# Autodesk Inventor assembly: 横回転ユニット改
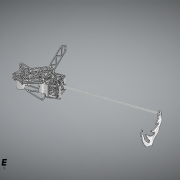
[picture p0: Inventor's stored thumbnail of the model, 180x180]
Saved by Autodesk Inventor 2020 (Build 240168000, 168)
## iProperties
Created: 2020-02-25
Part Number: 横回転ユニット改
Document SubType Name: Assembly
Designer: tanjihayato
Mass: 802.407 g
Surface Area: 1513.59 cm^2
Volume: 280.792 cm^3
Density: 2.85766 g/cm^3
Author: tanjihayato
## Documents named in this file (29)
- \\Mac\Home\Documents\Inventor\2019お遊び機体\横回転ユニット改.iam
- \\Mac\Home\Documents\Inventor\2019お遊び機体\横回転フレーム改.ipt
- \\Mac\Home\Documents\Inventor\2019お遊び機体\横回転フレーム改２.ipt
- \\Mac\Home\Documents\Inventor\2019お遊び機体\横回転フレーム改３.ipt
- \\Mac\Home\Documents\Inventor\2019お遊び機体\スペーサ　m3-l20.ipt
- \\Mac\Home\Documents\Inventor\2019お遊び機体\スペーサ　m3-l30.ipt
- \\Mac\Home\Documents\Inventor\2019お遊び機体\スペーサ　m3-l7.ipt
- \\Mac\Home\Documents\Inventor\2019お遊び機体\モーター(形だけ).ipt
- \\Mac\Home\Documents\Inventor\2019お遊び機体\横回転最終段.ipt
- \\Mac\Home\Documents\Inventor\2019お遊び機体\横回転最終段カム.ipt
- \\Mac\Home\Documents\Inventor\2019お遊び機体\横回転棒取り付けパーツ.ipt
- \\Mac\Home\Documents\Inventor\2019お遊び機体\横回転スライダー.ipt
- \\Mac\Home\Documents\Inventor\2019お遊び機体\ねじ皿　m3-l8.ipt
- \\Mac\Home\Documents\Inventor\2019お遊び機体\横回転フランジ付き軸.ipt
- \\Mac\Home\Documents\Inventor\2019お遊び機体\横回転シャフト.ipt
- \\Mac\Home\Documents\Inventor\2019お遊び機体\横回転フレーム改横.ipt
- \\Mac\Home\Documents\Inventor\2019お遊び機体\スペーサ　m3-l55.ipt
- \\Mac\Home\Documents\Inventor\2019お遊び機体\横回転首振りフレーム.ipt
- \\Mac\Home\Documents\Inventor\2019お遊び機体\横回転首振りフレーム２.ipt
- \\Mac\Home\Documents\Inventor\2019お遊び機体\スペーサ　m3-l12.ipt
- \\Mac\Home\Documents\Inventor\2019お遊び機体\アーム下板.ipt
- \\Mac\Home\Documents\Inventor\2019お遊び機体\スペーサ　m4-l45.ipt
- \\Mac\Home\Documents\Inventor\2019お遊び機体\横回転首振り駆動.ipt
- \\Mac\Home\Documents\Inventor\2019お遊び機体\フランジブッシュ　d8-D10-l5-f16.ipt
- \\Mac\Home\Documents\Inventor\2019お遊び機体\横回転鎌.ipt
- \\Mac\Home\Documents\Inventor\2019お遊び機体\m2z25.ipt
- \\Mac\Home\Documents\Inventor\2019お遊び機体\横回転首振り最終段カム.ipt
- \\Mac\Home\Documents\Inventor\2019お遊び機体\横回転カウンター根本.ipt
- \\Mac\Home\Documents\Inventor\2019お遊び機体\横回転首振りフレーム３.ipt
## Components (49 placed, 28 different names)
1. 横回転フレーム改:1 — 挿入:1, 挿入:2, 挿入:3, 挿入:4, 挿入:9, 挿入:10, 挿入:11, 挿入:12
2. 横回転フレーム改２:1 — 挿入:5, メイト:1, 挿入:7, 挿入:8, 挿入:14, メイト:3, メイト:4, メイト:5, メイト:6, メイト:7
3. 横回転フレーム改３:1 — 挿入:13, メイト:2
4. スペーサ　m3-l20:2 — 挿入:2, メイト:1
5. スペーサ　m3-l20:4 — 挿入:1, 挿入:5
6. スペーサ　m3-l30:1 — 挿入:4, メイト:2
7. スペーサ　m3-l30:2 — 挿入:3, 挿入:13
8. スペーサ　m3-l7:1 — 挿入:7
9. スペーサ　m3-l7:2 — 挿入:8
10. モーター(形だけ):1 — 挿入:9
11. モーター(形だけ):2 — 挿入:10
12. モーター(形だけ):3 — 挿入:11
13. モーター(形だけ):4 — 挿入:12
14. 横回転最終段:1 — 挿入:15, 挿入:23
15. 横回転最終段カム:1 — 挿入:14, メイト:3, 挿入:15, 挿入:16, 挿入:17, 挿入:25
16. 横回転棒取り付けパーツ:1 — 挿入:21, 挿入:22, 挿入:26
17. 横回転スライダー:1 — 挿入:21, 挿入:22, 挿入:24
18. ねじ皿　m3-l8:1 — 挿入:16
19. ねじ皿　m3-l8:2 — 挿入:17
20. 横回転フランジ付き軸:1 — 挿入:23, 挿入:24
21. 横回転フランジ付き軸:2 — 挿入:25
22. 横回転シャフト:1 — 挿入:26, 挿入:44
23. 横回転フレーム改横:1 — メイト:4, メイト:5
24. 横回転フレーム改横:2 — メイト:6, メイト:7, 挿入:27, 挿入:28, 挿入:29, 挿入:30, 挿入:42
25. スペーサ　m3-l55:1 — 挿入:30
26. スペーサ　m3-l55:2 — 挿入:29
27. スペーサ　m3-l55:3 — 挿入:27
28. スペーサ　m3-l55:4 — 挿入:28
29. 横回転首振りフレーム:1 — 挿入:35, メイト:11, 挿入:37, 挿入:38, 挿入:39, 挿入:40, 挿入:41, メイト:16, メイト:17, 挿入:47
30. 横回転首振りフレーム２:1 — メイト:8, メイト:9, メイト:10, 挿入:31, 挿入:32, 挿入:33, 挿入:34, 挿入:36, メイト:18, 挿入:48
31. スペーサ　m3-l12:1 — 挿入:33
32. スペーサ　m3-l12:2 — 挿入:31
33. スペーサ　m3-l12:3 — 挿入:34, 挿入:35
34. スペーサ　m3-l12:4 — 挿入:32, メイト:11
35. アーム下板:1 — メイト:8, メイト:9, メイト:10
36. スペーサ　m4-l45:1 — 挿入:36, メイト:12
37. スペーサ　m4-l45:2 — 挿入:38
38. スペーサ　m4-l45:3 — 挿入:37
39. モーター(形だけ):5 — 挿入:39
40. モーター(形だけ):6 — 挿入:40
41. 横回転首振り駆動:1 — 挿入:41, メイト:13, 挿入:43, 挿入:45, メイト:14
42. フランジブッシュ　d8-D10-l5-f16:1 — メイト:12, メイト:13
43. フランジブッシュ　d8-D10-l5-f16:2 — 挿入:42, 挿入:43
44. 横回転鎌:1 — 挿入:44
45. m2z25:1 — 挿入:46, メイト:15
46. 横回転首振り最終段カム:1 — 挿入:45, メイト:14, 挿入:46, メイト:15
47. 横回転カウンター根本:1 — メイト:16, メイト:17
48. 横回転首振りフレーム３:1 — 挿入:47, メイト:18
49. スペーサ　m3-l12:5 — 挿入:48
## Relationships (62: Insert 44, Mate 18)
- 挿入:1 [Insert]: 横回転フレーム改:1 ↔ スペーサ　m3-l20:4
- 挿入:2 [Insert]: 横回転フレーム改:1 ↔ スペーサ　m3-l20:2
- 挿入:3 [Insert]: 横回転フレーム改:1 ↔ スペーサ　m3-l30:2
- 挿入:4 [Insert]: 横回転フレーム改:1 ↔ スペーサ　m3-l30:1
- 挿入:5 [Insert]: 横回転フレーム改２:1 ↔ スペーサ　m3-l20:4
- メイト:1 [Mate]: 横回転フレーム改２:1 ↔ スペーサ　m3-l20:2
- 挿入:7 [Insert]: 横回転フレーム改２:1 ↔ スペーサ　m3-l7:1
- 挿入:8 [Insert]: 横回転フレーム改２:1 ↔ スペーサ　m3-l7:2
- 挿入:9 [Insert]: 横回転フレーム改:1 ↔ モーター(形だけ):1
- 挿入:10 [Insert]: 横回転フレーム改:1 ↔ モーター(形だけ):2
- 挿入:11 [Insert]: 横回転フレーム改:1 ↔ モーター(形だけ):3
- 挿入:12 [Insert]: 横回転フレーム改:1 ↔ モーター(形だけ):4
- 挿入:13 [Insert]: 横回転フレーム改３:1 ↔ スペーサ　m3-l30:2
- メイト:2 [Mate]: 横回転フレーム改３:1 ↔ スペーサ　m3-l30:1
- 挿入:14 [Insert]: 横回転フレーム改２:1 ↔ 横回転最終段カム:1
- メイト:3 [Mate]: 横回転フレーム改２:1 ↔ 横回転最終段カム:1
- 挿入:15 [Insert] (0.5 mm): 横回転最終段:1 ↔ 横回転最終段カム:1
- 挿入:16 [Insert]: 横回転最終段カム:1 ↔ ねじ皿　m3-l8:1
- 挿入:17 [Insert]: 横回転最終段カム:1 ↔ ねじ皿　m3-l8:2
- 挿入:21 [Insert]: 横回転棒取り付けパーツ:1 ↔ 横回転スライダー:1
- 挿入:22 [Insert]: 横回転棒取り付けパーツ:1 ↔ 横回転スライダー:1
- 挿入:23 [Insert]: 横回転最終段:1 ↔ 横回転フランジ付き軸:1
- 挿入:24 [Insert]: 横回転スライダー:1 ↔ 横回転フランジ付き軸:1
- 挿入:25 [Insert]: 横回転最終段カム:1 ↔ 横回転フランジ付き軸:2
- 挿入:26 [Insert]: 横回転棒取り付けパーツ:1 ↔ 横回転シャフト:1
- メイト:4 [Mate]: 横回転フレーム改２:1 ↔ 横回転フレーム改横:1
- メイト:5 [Mate]: 横回転フレーム改２:1 ↔ 横回転フレーム改横:1
- メイト:6 [Mate]: 横回転フレーム改２:1 ↔ 横回転フレーム改横:2
- メイト:7 [Mate]: 横回転フレーム改２:1 ↔ 横回転フレーム改横:2
- 挿入:27 [Insert]: 横回転フレーム改横:2 ↔ スペーサ　m3-l55:3
- 挿入:28 [Insert]: 横回転フレーム改横:2 ↔ スペーサ　m3-l55:4
- 挿入:29 [Insert]: 横回転フレーム改横:2 ↔ スペーサ　m3-l55:2
- 挿入:30 [Insert]: 横回転フレーム改横:2 ↔ スペーサ　m3-l55:1
- メイト:8 [Mate]: 横回転首振りフレーム２:1 ↔ アーム下板:1
- メイト:9 [Mate]: 横回転首振りフレーム２:1 ↔ アーム下板:1
- メイト:10 [Mate]: 横回転首振りフレーム２:1 ↔ アーム下板:1
- 挿入:31 [Insert]: 横回転首振りフレーム２:1 ↔ スペーサ　m3-l12:2
- 挿入:32 [Insert]: 横回転首振りフレーム２:1 ↔ スペーサ　m3-l12:4
- 挿入:33 [Insert]: 横回転首振りフレーム２:1 ↔ スペーサ　m3-l12:1
- 挿入:34 [Insert]: 横回転首振りフレーム２:1 ↔ スペーサ　m3-l12:3
- 挿入:35 [Insert]: 横回転首振りフレーム:1 ↔ スペーサ　m3-l12:3
- メイト:11 [Mate]: 横回転首振りフレーム:1 ↔ スペーサ　m3-l12:4
- 挿入:36 [Insert]: 横回転首振りフレーム２:1 ↔ スペーサ　m4-l45:1
- 挿入:37 [Insert]: 横回転首振りフレーム:1 ↔ スペーサ　m4-l45:3
- 挿入:38 [Insert]: 横回転首振りフレーム:1 ↔ スペーサ　m4-l45:2
- 挿入:39 [Insert]: 横回転首振りフレーム:1 ↔ モーター(形だけ):5
- 挿入:40 [Insert]: 横回転首振りフレーム:1 ↔ モーター(形だけ):6
- 挿入:41 [Insert] (0.5 mm): 横回転首振りフレーム:1 ↔ 横回転首振り駆動:1
- 挿入:42 [Insert]: 横回転フレーム改横:2 ↔ フランジブッシュ　d8-D10-l5-f16:2
- メイト:12 [Mate]: スペーサ　m4-l45:1 ↔ フランジブッシュ　d8-D10-l5-f16:1
- メイト:13 [Mate]: 横回転首振り駆動:1 ↔ フランジブッシュ　d8-D10-l5-f16:1
- 挿入:43 [Insert]: 横回転首振り駆動:1 ↔ フランジブッシュ　d8-D10-l5-f16:2
- 挿入:44 [Insert]: 横回転シャフト:1 ↔ 横回転鎌:1
- 挿入:45 [Insert]: 横回転首振り駆動:1 ↔ 横回転首振り最終段カム:1
- メイト:14 [Mate]: 横回転首振り駆動:1 ↔ 横回転首振り最終段カム:1
- 挿入:46 [Insert]: m2z25:1 ↔ 横回転首振り最終段カム:1
- メイト:15 [Mate]: m2z25:1 ↔ 横回転首振り最終段カム:1
- メイト:16 [Mate]: 横回転首振りフレーム:1 ↔ 横回転カウンター根本:1
- メイト:17 [Mate]: 横回転首振りフレーム:1 ↔ 横回転カウンター根本:1
- 挿入:47 [Insert] (71 mm): 横回転首振りフレーム:1 ↔ 横回転首振りフレーム３:1
- メイト:18 [Mate]: 横回転首振りフレーム２:1 ↔ 横回転首振りフレーム３:1
- 挿入:48 [Insert]: 横回転首振りフレーム２:1 ↔ スペーサ　m3-l12:5
